# Autodesk Inventor assembly: DT Side Assembly_MIR
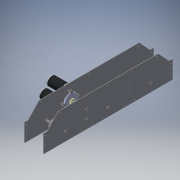
[picture p0: Inventor's stored thumbnail of the model, 180x180]
Saved by Autodesk Inventor 2016 (Build 200138000, 138)
## iProperties
Created: 2018-05-03
Part Number: DT Side Assembly_MIR
Document SubType Name: Assembly
Designer: Kade
Author: 2000083068
## Documents named in this file (12)
- F:\Robotics\Off Season\Blannon\DT Side Assembly_MIR.iam
- F:\Robotics\Off Season\Blannon\Fixed Side frame_MIR.ipt
- F:\Robotics\Off Season\Blannon\.5 ID Flanged Bearing_MIR.ipt
- F:\Robotics\Off Season\Blannon\ThunderHex_Stock_18in_MIR.ipt
- F:\Robotics\Off Season\Blannon\72t_Aluminum_Spur_Gear_20_DP_1_2_Hex_Bore_217-3576_MIR.ipt
- F:\Robotics\Off Season\Blannon\24t_Steel_Spur_Gear_20_DP_1_2_Hex_Bore_217-5464_MIR.ipt
- F:\Robotics\Off Season\Blannon\Cim Motor_MIR.ipt
- F:\Robotics\Off Season\Blannon\11t_Steel_Spur_Gear_20_DP_CIM_Motor_12t_Center_Distance_217-3107_MIR.ipt
- F:\Robotics\Off Season\Blannon\Wheel Hub_MIR.ipt
- F:\Robotics\Off Season\Blannon\36t_x_15mm_Wide_Aluminum_Pulley_HTD_5mm_1_2_Hex_217-4103_MIR.ipt
- F:\Robotics\Off Season\Blannon\36t_x_9mm_Wide_Double_Flange_Aluminum_Pulley_HTD_5mm_1_2_Hex_Bore_217-3231_MIR.ipt
- F:\Robotics\Off Season\Blannon\Fixed Side Frame Outside_MIR.ipt
## Components (33 placed, 11 different names)
1. Fixed Side frame_MIR:1 — Mate:39, Mate:3, Mate:2, Mate:12, Mate:6, Mate:15, Mate:4, Mate:41, Mate:7, Mate:40, Mate:8, Mate:42, Mate:5, Mate:25, Mate:21, Mate:24, Mate:22, Mate:23, Mate:20, Mate:65, Flush:15, Flush:14
2. .5 ID Flanged Bearing_MIR:1 — Mate:12, Mate:6, Mate:13, Flush:1, Mate:14
3. .5 ID Flanged Bearing_MIR:2 — Mate:15, Mate:4, Flush:2, Mate:10
4. .5 ID Flanged Bearing_MIR:3 — Mate:41, Mate:7, Flush:4, Mate:33
5. .5 ID Flanged Bearing_MIR:4 — Mate:40, Mate:8, Flush:3, Mate:32
6. .5 ID Flanged Bearing_MIR:5 — Mate:42, Mate:5, Flush:5, Mate:34
7. ThunderHex_Stock_18in_MIR:1 — Mate:13, Flush:1, Mate:11, Mate:18
8. ThunderHex_Stock_18in_MIR:2 — Flush:2, Mate:10, Mate:16, Mate:58, Mate:57
9. 72t_Aluminum_Spur_Gear_20_DP_1_2_Hex_Bore_217-3576_MIR:1 — Mate:14, Mate:11, Mate:19
10. 72t_Aluminum_Spur_Gear_20_DP_1_2_Hex_Bore_217-3576_MIR:2 — Mate:16, Flush:9, Mate:59, Mate:64
11. 24t_Steel_Spur_Gear_20_DP_1_2_Hex_Bore_217-5464_MIR:1 — Flush:9, Mate:19, Mate:18
12. Cim Motor_MIR:1 — Mate:25, Mate:21, Flush:8, Mate:31
13. Cim Motor_MIR:2 — Mate:24, Mate:22, Flush:6, Mate:29
14. Cim Motor_MIR:3 — Mate:23, Mate:20, Flush:7, Mate:30
15. 11t_Steel_Spur_Gear_20_DP_CIM_Motor_12t_Center_Distance_217-3107_MIR:1 — Flush:6, Mate:29
16. 11t_Steel_Spur_Gear_20_DP_CIM_Motor_12t_Center_Distance_217-3107_MIR:2 — Flush:8, Mate:31
17. 11t_Steel_Spur_Gear_20_DP_CIM_Motor_12t_Center_Distance_217-3107_MIR:3 — Flush:7, Mate:30
18. ThunderHex_Stock_18in_MIR:3 — Flush:4, Mate:33, Mate:44, Mate:54, Mate:53
19. ThunderHex_Stock_18in_MIR:4 — Flush:3, Mate:32, Mate:43, Mate:61, Mate:60
20. ThunderHex_Stock_18in_MIR:5 — Flush:5, Mate:34, Mate:50, Mate:63, Mate:62
21. Wheel Hub_MIR:1 — Mate:43, Flush:12
22. Wheel Hub_MIR:2 — Flush:12, Mate:44, Flush:13, Mate:56
23. Wheel Hub_MIR:3 — Flush:13, Mate:50
24. 36t_x_15mm_Wide_Aluminum_Pulley_HTD_5mm_1_2_Hex_217-4103_MIR:1 — Mate:59, Mate:58, Mate:57, Flush:10
25. 36t_x_15mm_Wide_Aluminum_Pulley_HTD_5mm_1_2_Hex_217-4103_MIR:2 — Flush:10, Mate:56, Mate:54, Mate:53, Flush:11
26. 36t_x_9mm_Wide_Double_Flange_Aluminum_Pulley_HTD_5mm_1_2_Hex_Bore_217-3231_MIR:1 — Flush:11, Mate:61, Mate:60
27. 36t_x_9mm_Wide_Double_Flange_Aluminum_Pulley_HTD_5mm_1_2_Hex_Bore_217-3231_MIR:2 — Mate:64, Mate:63, Mate:62
28. .5 ID Flanged Bearing_MIR:6
29. .5 ID Flanged Bearing_MIR:7
30. .5 ID Flanged Bearing_MIR:8
31. .5 ID Flanged Bearing_MIR:9
32. .5 ID Flanged Bearing_MIR:10
33. Fixed Side Frame Outside_MIR:1 — Mate:65, Flush:15, Flush:14
## Relationships (62: Mate 47, Flush 15)
- Mate:39: Fixed Side frame_MIR:1
- Mate:3: Fixed Side frame_MIR:1
- Mate:2 (127 mm): Fixed Side frame_MIR:1
- Mate:12: Fixed Side frame_MIR:1 ↔ .5 ID Flanged Bearing_MIR:1
- Mate:6 (-3.175 mm): Fixed Side frame_MIR:1 ↔ .5 ID Flanged Bearing_MIR:1
- Mate:15: Fixed Side frame_MIR:1 ↔ .5 ID Flanged Bearing_MIR:2
- Mate:4 (-3.175 mm): Fixed Side frame_MIR:1 ↔ .5 ID Flanged Bearing_MIR:2
- Mate:41: Fixed Side frame_MIR:1 ↔ .5 ID Flanged Bearing_MIR:3
- Mate:7 (-3.175 mm): Fixed Side frame_MIR:1 ↔ .5 ID Flanged Bearing_MIR:3
- Mate:40: Fixed Side frame_MIR:1 ↔ .5 ID Flanged Bearing_MIR:4
- Mate:8 (-3.175 mm): Fixed Side frame_MIR:1 ↔ .5 ID Flanged Bearing_MIR:4
- Mate:42: Fixed Side frame_MIR:1 ↔ .5 ID Flanged Bearing_MIR:5
- Mate:5 (-6.35 mm): Fixed Side frame_MIR:1 ↔ .5 ID Flanged Bearing_MIR:5
- Mate:13: .5 ID Flanged Bearing_MIR:1 ↔ ThunderHex_Stock_18in_MIR:1
- Flush:1: .5 ID Flanged Bearing_MIR:1 ↔ ThunderHex_Stock_18in_MIR:1
- Flush:2: .5 ID Flanged Bearing_MIR:2 ↔ ThunderHex_Stock_18in_MIR:2
- Mate:10: .5 ID Flanged Bearing_MIR:2 ↔ ThunderHex_Stock_18in_MIR:2
- Mate:14 (8.89 mm): .5 ID Flanged Bearing_MIR:1 ↔ 72t_Aluminum_Spur_Gear_20_DP_1_2_Hex_Bore_217-3576_MIR:1
- Mate:11: ThunderHex_Stock_18in_MIR:1 ↔ 72t_Aluminum_Spur_Gear_20_DP_1_2_Hex_Bore_217-3576_MIR:1
- Mate:16: ThunderHex_Stock_18in_MIR:2 ↔ 72t_Aluminum_Spur_Gear_20_DP_1_2_Hex_Bore_217-3576_MIR:2
- Flush:9 (-1.27 mm): 72t_Aluminum_Spur_Gear_20_DP_1_2_Hex_Bore_217-3576_MIR:2 ↔ 24t_Steel_Spur_Gear_20_DP_1_2_Hex_Bore_217-5464_MIR:1
- Mate:19: 72t_Aluminum_Spur_Gear_20_DP_1_2_Hex_Bore_217-3576_MIR:1 ↔ 24t_Steel_Spur_Gear_20_DP_1_2_Hex_Bore_217-5464_MIR:1
- Mate:18: ThunderHex_Stock_18in_MIR:1 ↔ 24t_Steel_Spur_Gear_20_DP_1_2_Hex_Bore_217-5464_MIR:1
- Mate:25: Fixed Side frame_MIR:1 ↔ Cim Motor_MIR:1
- Mate:21: Fixed Side frame_MIR:1 ↔ Cim Motor_MIR:1
- Mate:24: Fixed Side frame_MIR:1 ↔ Cim Motor_MIR:2
- Mate:22: Fixed Side frame_MIR:1 ↔ Cim Motor_MIR:2
- Mate:23: Fixed Side frame_MIR:1 ↔ Cim Motor_MIR:3
- Mate:20: Fixed Side frame_MIR:1 ↔ Cim Motor_MIR:3
- Flush:6: Cim Motor_MIR:2 ↔ 11t_Steel_Spur_Gear_20_DP_CIM_Motor_12t_Center_Distance_217-3107_MIR:1
- Mate:29: Cim Motor_MIR:2 ↔ 11t_Steel_Spur_Gear_20_DP_CIM_Motor_12t_Center_Distance_217-3107_MIR:1
- Flush:8: Cim Motor_MIR:1 ↔ 11t_Steel_Spur_Gear_20_DP_CIM_Motor_12t_Center_Distance_217-3107_MIR:2
- Mate:31: Cim Motor_MIR:1 ↔ 11t_Steel_Spur_Gear_20_DP_CIM_Motor_12t_Center_Distance_217-3107_MIR:2
- Flush:7: Cim Motor_MIR:3 ↔ 11t_Steel_Spur_Gear_20_DP_CIM_Motor_12t_Center_Distance_217-3107_MIR:3
- Mate:30: Cim Motor_MIR:3 ↔ 11t_Steel_Spur_Gear_20_DP_CIM_Motor_12t_Center_Distance_217-3107_MIR:3
- Flush:4: .5 ID Flanged Bearing_MIR:3 ↔ ThunderHex_Stock_18in_MIR:3
- Mate:33: .5 ID Flanged Bearing_MIR:3 ↔ ThunderHex_Stock_18in_MIR:3
- Flush:3: .5 ID Flanged Bearing_MIR:4 ↔ ThunderHex_Stock_18in_MIR:4
- Mate:32: .5 ID Flanged Bearing_MIR:4 ↔ ThunderHex_Stock_18in_MIR:4
- Flush:5: .5 ID Flanged Bearing_MIR:5 ↔ ThunderHex_Stock_18in_MIR:5
- Mate:34: .5 ID Flanged Bearing_MIR:5 ↔ ThunderHex_Stock_18in_MIR:5
- Mate:43: ThunderHex_Stock_18in_MIR:4 ↔ Wheel Hub_MIR:1
- Flush:12: Wheel Hub_MIR:1 ↔ Wheel Hub_MIR:2
- Mate:44: ThunderHex_Stock_18in_MIR:3 ↔ Wheel Hub_MIR:2
- Flush:13: Wheel Hub_MIR:2 ↔ Wheel Hub_MIR:3
- Mate:50: ThunderHex_Stock_18in_MIR:5 ↔ Wheel Hub_MIR:3
- Mate:59: 72t_Aluminum_Spur_Gear_20_DP_1_2_Hex_Bore_217-3576_MIR:2 ↔ 36t_x_15mm_Wide_Aluminum_Pulley_HTD_5mm_1_2_Hex_217-4103_MIR:1
- Mate:58: ThunderHex_Stock_18in_MIR:2 ↔ 36t_x_15mm_Wide_Aluminum_Pulley_HTD_5mm_1_2_Hex_217-4103_MIR:1
- Mate:57: ThunderHex_Stock_18in_MIR:2 ↔ 36t_x_15mm_Wide_Aluminum_Pulley_HTD_5mm_1_2_Hex_217-4103_MIR:1
- Flush:10: 36t_x_15mm_Wide_Aluminum_Pulley_HTD_5mm_1_2_Hex_217-4103_MIR:1 ↔ 36t_x_15mm_Wide_Aluminum_Pulley_HTD_5mm_1_2_Hex_217-4103_MIR:2
- Mate:56 (12.7 mm): Wheel Hub_MIR:2 ↔ 36t_x_15mm_Wide_Aluminum_Pulley_HTD_5mm_1_2_Hex_217-4103_MIR:2
- Mate:54: ThunderHex_Stock_18in_MIR:3 ↔ 36t_x_15mm_Wide_Aluminum_Pulley_HTD_5mm_1_2_Hex_217-4103_MIR:2
- Mate:53: ThunderHex_Stock_18in_MIR:3 ↔ 36t_x_15mm_Wide_Aluminum_Pulley_HTD_5mm_1_2_Hex_217-4103_MIR:2
- Flush:11: 36t_x_15mm_Wide_Aluminum_Pulley_HTD_5mm_1_2_Hex_217-4103_MIR:2 ↔ 36t_x_9mm_Wide_Double_Flange_Aluminum_Pulley_HTD_5mm_1_2_Hex_Bore_217-3231_MIR:1
- Mate:61: ThunderHex_Stock_18in_MIR:4 ↔ 36t_x_9mm_Wide_Double_Flange_Aluminum_Pulley_HTD_5mm_1_2_Hex_Bore_217-3231_MIR:1
- Mate:60: ThunderHex_Stock_18in_MIR:4 ↔ 36t_x_9mm_Wide_Double_Flange_Aluminum_Pulley_HTD_5mm_1_2_Hex_Bore_217-3231_MIR:1
- Mate:64: 72t_Aluminum_Spur_Gear_20_DP_1_2_Hex_Bore_217-3576_MIR:2 ↔ 36t_x_9mm_Wide_Double_Flange_Aluminum_Pulley_HTD_5mm_1_2_Hex_Bore_217-3231_MIR:2
- Mate:63: ThunderHex_Stock_18in_MIR:5 ↔ 36t_x_9mm_Wide_Double_Flange_Aluminum_Pulley_HTD_5mm_1_2_Hex_Bore_217-3231_MIR:2
- Mate:62: ThunderHex_Stock_18in_MIR:5 ↔ 36t_x_9mm_Wide_Double_Flange_Aluminum_Pulley_HTD_5mm_1_2_Hex_Bore_217-3231_MIR:2
- Mate:65 (132.334 mm): Fixed Side frame_MIR:1 ↔ Fixed Side Frame Outside_MIR:1
- Flush:15: Fixed Side frame_MIR:1 ↔ Fixed Side Frame Outside_MIR:1
- Flush:14: Fixed Side frame_MIR:1 ↔ Fixed Side Frame Outside_MIR:1
